# Autodesk Inventor assembly: Assembly6_arm
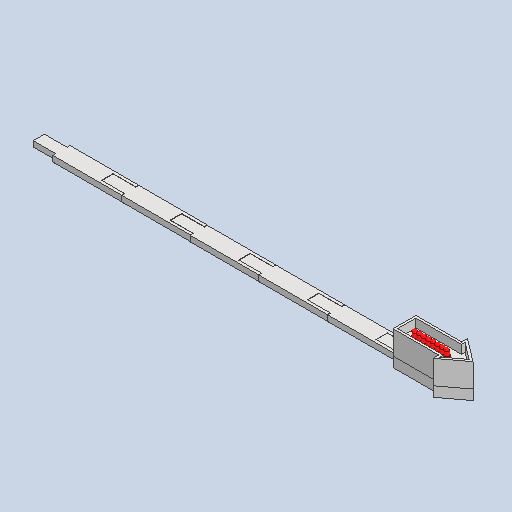
[picture p0: Inventor's stored thumbnail of the model, 512x512]
Saved by Autodesk Inventor 2023 (Build 270158000, 158)
## iProperties
Created: 2023-10-25
Part Number: Assembly6_arm
Document SubType Name: Assembly
Designer: zskus
Author: zskus
## Documents named in this file (4)
- C:\Users\zskus\Desktop\Folders\Personal Projects\Inventor\Project_1_Scooter\Assembly\Assembly6_arm.iam
- C:\Users\zskus\Desktop\Folders\Personal Projects\Inventor\Project_1_Scooter\Assembly\Assembly5_turnsignal_back.iam
- C:\Users\zskus\Desktop\Folders\Personal Projects\Inventor\Project_1_Scooter\Assembly\Assembly_4_turnsignal_MIR.iam
- C:\Users\zskus\Desktop\Folders\Personal Projects\Inventor\Project_1_Scooter\Parts\Part_3_hand_extention.ipt
## Components (7 placed, 3 different names)
1. Assembly5_turnsignal_back:1 [sub-assembly] — Mate:1, Flush:1, Flush:2
2. Assembly_4_turnsignal_MIR:1 [sub-assembly] — Mate:1, Flush:1, Flush:2, Mate:2, Mate:3, Mate:4
3. Part_3_hand_extention:1 — Mate:2, Mate:3, Mate:4, Mate:5, Mate:6, Mate:7
4. Part_3_hand_extention:2 — Mate:5, Mate:6, Mate:7, Mate:8, Mate:9, Mate:10
5. Part_3_hand_extention:3 — Mate:8, Mate:9, Mate:10, Mate:11, Mate:12, Mate:13
6. Part_3_hand_extention:4 — Mate:11, Mate:12, Mate:13, Mate:14, Mate:15, Mate:16
7. Part_3_hand_extention:5 — Mate:14, Mate:15, Mate:16
## Relationships (18: Mate 16, Flush 2)
- Mate:1: Assembly5_turnsignal_back:1 ↔ Assembly_4_turnsignal_MIR:1
- Flush:1: Assembly5_turnsignal_back:1 ↔ Assembly_4_turnsignal_MIR:1
- Flush:2: Assembly5_turnsignal_back:1 ↔ Assembly_4_turnsignal_MIR:1
- Mate:2: Assembly_4_turnsignal_MIR:1 ↔ Part_3_hand_extention:1
- Mate:3: Assembly_4_turnsignal_MIR:1 ↔ Part_3_hand_extention:1
- Mate:4: Assembly_4_turnsignal_MIR:1 ↔ Part_3_hand_extention:1
- Mate:5: Part_3_hand_extention:1 ↔ Part_3_hand_extention:2
- Mate:6: Part_3_hand_extention:1 ↔ Part_3_hand_extention:2
- Mate:7: Part_3_hand_extention:1 ↔ Part_3_hand_extention:2
- Mate:8: Part_3_hand_extention:2 ↔ Part_3_hand_extention:3
- Mate:9: Part_3_hand_extention:2 ↔ Part_3_hand_extention:3
- Mate:10: Part_3_hand_extention:2 ↔ Part_3_hand_extention:3
- Mate:11: Part_3_hand_extention:3 ↔ Part_3_hand_extention:4
- Mate:12: Part_3_hand_extention:3 ↔ Part_3_hand_extention:4
- Mate:13: Part_3_hand_extention:3 ↔ Part_3_hand_extention:4
- Mate:14: Part_3_hand_extention:4 ↔ Part_3_hand_extention:5
- Mate:15: Part_3_hand_extention:4 ↔ Part_3_hand_extention:5
- Mate:16: Part_3_hand_extention:4 ↔ Part_3_hand_extention:5
